# Autodesk Inventor assembly: UA-70 Denkmal
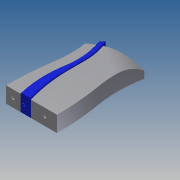
[picture p0: Inventor's stored thumbnail of the model, 180x180]
Saved by Autodesk Inventor 2014 SP2 (Build 180246200, 246)
## iProperties
Created: 2014-07-02
Part Number: UA-70 Denkmal
Document SubType Name: Assembly
Designer: Semenov
Author: Semenov
## Documents named in this file (3)
- W:\DATEN_INVENTOR\LiTHOS_FORMEN\UA\UA-070\UA-070 100x100\UA-70 Denkmal.iam
- W:\DATEN_INVENTOR\LiTHOS_FORMEN\UA\UA-070\UA-070 100x100\UA-70 Denkmal1.ipt
- W:\DATEN_INVENTOR\LiTHOS_FORMEN\UA\UA-070\UA-070 100x100\UA-70 Denkmal2.ipt
## Components (2 placed, 2 different names)
1. UA-70 Denkmal1:1 — Fluchtend:1, Fluchtend:2, Fluchtend:3
2. UA-70 Denkmal2:1 — Fluchtend:1, Fluchtend:2, Fluchtend:3
## Relationships (3: Flush 3)
- Fluchtend:1 [Flush]: UA-70 Denkmal1:1 ↔ UA-70 Denkmal2:1
- Fluchtend:2 [Flush]: UA-70 Denkmal1:1 ↔ UA-70 Denkmal2:1
- Fluchtend:3 [Flush]: UA-70 Denkmal1:1 ↔ UA-70 Denkmal2:1
